# Autodesk Inventor assembly: final assembly
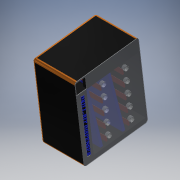
[picture p0: Inventor's stored thumbnail of the model, 180x180]
Saved by Autodesk Inventor 2019 (Build 230136000, 136)
## iProperties
Created: 2020-03-10
Part Number: final assembly
Document SubType Name: Assembly
Designer: Hp
Author: Hp
## Documents named in this file (4)
- F:\2nd sem\INVENTOR\KSHITEJ\final assembly.iam
- F:\2nd sem\INVENTOR\KSHITEJ\step motor.ipt
- F:\2nd sem\INVENTOR\KSHITEJ\OUTER CASE.ipt
- F:\2nd sem\INVENTOR\KSHITEJ\frount glass.ipt
## Components (12 placed, 3 different names)
1. OUTER CASE:1 — Rigid:1, Rigid:2
2. frount glass:1 — Rigid:2
3. step motor:3 — Rigid:1
4. step motor:11
5. step motor:12
6. step motor:13
7. step motor:14
8. step motor:15
9. step motor:16
10. step motor:17
11. step motor:18
12. step motor:19
## Component patterns: (2 elements), (5 elements, first: step motor:3), Component Pattern 1:2 (5 elements)
## Relationships (2: WeldJoint 2)
- Rigid:1 [WeldJoint]: OUTER CASE:1 ↔ step motor:3
- Rigid:2 [WeldJoint]: OUTER CASE:1 ↔ frount glass:1
